# Autodesk Inventor assembly: canaletaVar
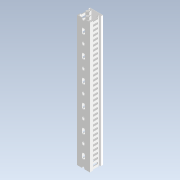
[picture p0: Inventor's stored thumbnail of the model, 180x180]
Saved by Autodesk Inventor 2021 (Build 250183000, 183)
## iProperties
Created: 2021-08-23
Part Number: canaletaVar
Document SubType Name: Assembly
Designer: Andrés Holguín
Author: Andrés Holguín
## Documents named in this file (2)
- C:\Users\andre\Documents\GitHub\Dis.-Mecatronico-E6\inventor proyecto\Tablero\Canaletas\canaletaVar.iam
- C:\Users\andre\Documents\GitHub\Dis.-Mecatronico-E6\inventor proyecto\Tablero\Canaletas\7308-1.iam
## Components (2 placed, 1 different names)
1. 7308-1:1 [sub-assembly] — Rigid:1
2. 7308-1:2 [sub-assembly] — Rigid:1
## Relationships (1: WeldJoint 1)
- Rigid:1 [WeldJoint]: 7308-1:1 ↔ 7308-1:2
